# Autodesk Inventor assembly: Abdeckung_Gaseinlass
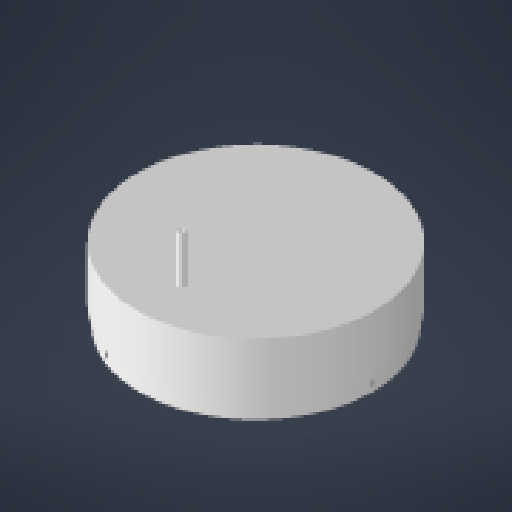
[picture p0: Inventor's stored thumbnail of the model, 512x512]
Saved by Autodesk Inventor 2027 (Build 310192060, 192F)
## iProperties
Created: 2026-08-01
Part Number: Abdeckung_Gaseinlass
Document SubType Name: Assembly
Designer: kw
Author: kw
## Documents named in this file (3)
- C:\Users\kw\OneDrive\Documents\Uni\Masterthesis\Spezialisierungsmodul\InventorZeichnungen_Konrad\4er-AktuellesDesign\Abdeckung_Gaseinlass.iam
- C:\Users\kw\OneDrive\Documents\Uni\Masterthesis\Spezialisierungsmodul\InventorZeichnungen_Konrad\4er-AktuellesDesign\Abdeckung_Gaseinlass_new.ipt
- C:\Users\kw\OneDrive\Documents\Uni\Masterthesis\Spezialisierungsmodul\InventorZeichnungen_Konrad\4er-AktuellesDesign\GasEinlass_Flansch.ipt
## Components (2 placed, 2 different names)
1. Abdeckung_Gaseinlass_new:1 — Mate:1, Flush:1
2. GasEinlass_Flansch:1 — Mate:1, Flush:1
## Relationships (2: Mate 1, Flush 1)
- Mate:1: Abdeckung_Gaseinlass_new:1 ↔ GasEinlass_Flansch:1
- Flush:1 (-9 mm): Abdeckung_Gaseinlass_new:1 ↔ GasEinlass_Flansch:1
